# Autodesk Inventor assembly: YAxis
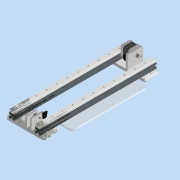
[picture p0: Inventor's stored thumbnail of the model, 180x180]
Saved by Autodesk Inventor 2022 (Build 260153000, 153)
## iProperties
Created: 2021-06-27
Part Number: YAxis
Document SubType Name: Assembly
Designer: domin
Author: domin
## Documents named in this file (19)
- D:\Sync\Hivemind\1-MCI-Unterlagen\Master\Semester 3\Projekt 2\011_Kartesischer_Roboter_Modul\07-CAD Files\02-Kartesischer Roboter\YAxis\YAxis.iam
- D:\Sync\Hivemind\1-MCI-Unterlagen\Master\Semester 3\Projekt 2\011_Kartesischer_Roboter_Modul\07-CAD Files\02-Kartesischer Roboter\Einzelteile\Fuehrungslager.ipt
- D:\Sync\Hivemind\1-MCI-Unterlagen\Master\Semester 3\Projekt 2\011_Kartesischer_Roboter_Modul\07-CAD Files\02-Kartesischer Roboter\Einzelteile\Y-Axis_back_plate_bottom.ipt
- D:\Sync\Hivemind\1-MCI-Unterlagen\Master\Semester 3\Projekt 2\011_Kartesischer_Roboter_Modul\07-CAD Files\02-Kartesischer Roboter\Einzelteile\Y-Axis_back_plate_top.ipt
- D:\Sync\Hivemind\1-MCI-Unterlagen\Master\Semester 3\Projekt 2\011_Kartesischer_Roboter_Modul\07-CAD Files\02-Kartesischer Roboter\Einzelteile\Y-Axis_front_plate_bottom.ipt
- D:\Sync\Hivemind\1-MCI-Unterlagen\Master\Semester 3\Projekt 2\011_Kartesischer_Roboter_Modul\07-CAD Files\02-Kartesischer Roboter\Einzelteile\Y-Axis_front_plate_top.ipt
- D:\Sync\Hivemind\1-MCI-Unterlagen\Master\Semester 3\Projekt 2\011_Kartesischer_Roboter_Modul\07-CAD Files\02-Kartesischer Roboter\Aluminum\X-Axis_motor_plate.ipt
- D:\Sync\Hivemind\1-MCI-Unterlagen\Master\Semester 3\Projekt 2\011_Kartesischer_Roboter_Modul\07-CAD Files\02-Kartesischer Roboter\Einzelteile\X-Kettenhalter2.ipt
- D:\Sync\Hivemind\1-MCI-Unterlagen\Master\Semester 3\Projekt 2\011_Kartesischer_Roboter_Modul\07-CAD Files\02-Kartesischer Roboter\Einzelteile\Y-Umlenkrollenhalter.ipt
- D:\Sync\Hivemind\1-MCI-Unterlagen\Master\Semester 3\Projekt 2\011_Kartesischer_Roboter_Modul\07-CAD Files\02-Kartesischer Roboter\Aluminum\X-Axis_beltplates.ipt
- D:\Sync\Hivemind\1-MCI-Unterlagen\Master\Semester 3\Projekt 2\011_Kartesischer_Roboter_Modul\07-CAD Files\02-Kartesischer Roboter\Einzelteile\Stift_5mm.ipt
- D:\Sync\Hivemind\1-MCI-Unterlagen\Master\Semester 3\Projekt 2\011_Kartesischer_Roboter_Modul\07-CAD Files\02-Kartesischer Roboter\Einzelteile\White_Cable_Tie_Mount_RS666-717.ipt
- D:\Sync\Hivemind\1-MCI-Unterlagen\Master\Semester 3\Projekt 2\011_Kartesischer_Roboter_Modul\07-CAD Files\02-Kartesischer Roboter\Einzelteile\Ender_Motor.ipt
- D:\Sync\Hivemind\1-MCI-Unterlagen\Master\Semester 3\Projekt 2\011_Kartesischer_Roboter_Modul\07-CAD Files\02-Kartesischer Roboter\Einzelteile\Endstop.ipt
- D:\Sync\Hivemind\1-MCI-Unterlagen\Master\Semester 3\Projekt 2\011_Kartesischer_Roboter_Modul\07-CAD Files\02-Kartesischer Roboter\Einzelteile\Umlenkrolle_5mm.ipt
- D:\Sync\Hivemind\1-MCI-Unterlagen\Master\Semester 3\Projekt 2\011_Kartesischer_Roboter_Modul\07-CAD Files\02-Kartesischer Roboter\Einzelteile\Zahnriemenscheibe_20teeth.ipt
- D:\Sync\Hivemind\1-MCI-Unterlagen\Master\Semester 3\Projekt 2\011_Kartesischer_Roboter_Modul\07-CAD Files\02-Kartesischer Roboter\ITEM_Profile\Schlitten_Profil.ipt
- D:\Sync\Hivemind\1-MCI-Unterlagen\Master\Semester 3\Projekt 2\011_Kartesischer_Roboter_Modul\07-CAD Files\02-Kartesischer Roboter\Einzelteile\Fuehrungsschiene440mm.ipt
- D:\Sync\Hivemind\1-MCI-Unterlagen\Master\Semester 3\Projekt 2\011_Kartesischer_Roboter_Modul\07-CAD Files\02-Kartesischer Roboter\Einzelteile\Y_Kettenhalter.ipt
## Components (25 placed, 18 different names)
1. Fuehrungslager:1 — Flush:2, Flush:3, Mate:1, Mate:2, Flush:4, Flush:5, Flush:6, Mate:3, Flush:7
2. Fuehrungslager:2 — Mate:2, Flush:4, Flush:5, Mate:5, Mate:6, Mate:7
3. Fuehrungslager:3 — Flush:6, Mate:3, Flush:7, Flush:8, Flush:9, Mate:4, Mate:9
4. Fuehrungslager:4 — Flush:8, Flush:9, Mate:4, Mate:10, Mate:11, Mate:47
5. Y-Axis_back_plate_bottom:1 — Mate:5, Mate:6, Mate:7, Mate:8, Flush:10, Flush:11
6. Y-Axis_back_plate_top:1 — Mate:8, Flush:10, Flush:11, Mate:13, Mate:14, Mate:15, Mate:16, Mate:17, Mate:18, Mate:40, Mate:42, Flush:17
7. Y-Axis_front_plate_bottom:1 — Mate:9, Mate:10, Mate:11, Mate:12, Flush:12, Flush:13
8. Y-Axis_front_plate_top:1 — Mate:12, Flush:12, Flush:13, Mate:19, Mate:20, Mate:21, Mate:22, Mate:23, Mate:24
9. X-Axis_motor_plate:1 — Mate:13, Mate:14, Mate:15, Mate:28, Mate:29, Mate:30, Mate:31, Mate:32, Mate:33, Flush:15
10. X-Kettenhalter2:1 — Mate:16, Mate:17, Mate:18, Mate:26, Mate:27, Angle:1, Mate:41
11. White_Cable_Tie_Mount_RS666-717:1 — Mate:26, Mate:27, Angle:1
12. Y-Umlenkrollenhalter:1 — Mate:19, Mate:20, Mate:21, Mate:25, Flush:14
13. X-Axis_beltplates:1 — Mate:22, Mate:23, Mate:24, Mate:34, Mate:36, Mate:37, Mate:38
14. Stift_5mm:1 — Mate:25, Flush:14, Mate:35
15. Ender_Motor:1 — Mate:28, Mate:29, Mate:30, Mate:39
16. Endstop:1 — Mate:31, Mate:32, Mate:33
17. Endstop:2 — Mate:36, Mate:37, Mate:38
18. Umlenkrolle_5mm:1 — Mate:34, Mate:35
19. Zahnriemenscheibe_20teeth:1 — Mate:39, Flush:15
20. Schlitten_Profil:1 — Mate:40, Mate:41, Mate:43, Flush:16, Flush:17, Mate:44, Flush:18, Flush:19, Mate:46, Flush:22, Mate:48, Mate:49
21. Schlitten_Profil:2 — Mate:42, Mate:43, Flush:16, Mate:45, Flush:20, Flush:21
22. Fuehrungsschiene440mm:1 — Mate:44, Flush:18, Flush:19
23. Fuehrungsschiene440mm:2 — Mate:45, Flush:20, Flush:21
24. Y_Kettenhalter:1 — Mate:46, Flush:22, Mate:47, Mate:50
25. White_Cable_Tie_Mount_RS666-717:2 — Mate:48, Mate:49, Mate:50
## Relationships (72: Mate 50, Flush 21, Angle 1)
- Flush:2: Fuehrungslager:1
- Flush:3: Fuehrungslager:1
- Mate:1: Fuehrungslager:1
- Mate:2 (36 mm): Fuehrungslager:1 ↔ Fuehrungslager:2
- Flush:4: Fuehrungslager:1 ↔ Fuehrungslager:2
- Flush:5: Fuehrungslager:1 ↔ Fuehrungslager:2
- Flush:6: Fuehrungslager:1 ↔ Fuehrungslager:3
- Mate:3 (358 mm): Fuehrungslager:1 ↔ Fuehrungslager:3
- Flush:7: Fuehrungslager:1 ↔ Fuehrungslager:3
- Flush:8: Fuehrungslager:3 ↔ Fuehrungslager:4
- Flush:9: Fuehrungslager:3 ↔ Fuehrungslager:4
- Mate:4 (36 mm): Fuehrungslager:3 ↔ Fuehrungslager:4
- Mate:5: Fuehrungslager:2 ↔ Y-Axis_back_plate_bottom:1
- Mate:6: Fuehrungslager:2 ↔ Y-Axis_back_plate_bottom:1
- Mate:7: Fuehrungslager:2 ↔ Y-Axis_back_plate_bottom:1
- Mate:8: Y-Axis_back_plate_bottom:1 ↔ Y-Axis_back_plate_top:1
- Flush:10: Y-Axis_back_plate_bottom:1 ↔ Y-Axis_back_plate_top:1
- Flush:11: Y-Axis_back_plate_bottom:1 ↔ Y-Axis_back_plate_top:1
- Mate:9: Fuehrungslager:3 ↔ Y-Axis_front_plate_bottom:1
- Mate:10: Fuehrungslager:4 ↔ Y-Axis_front_plate_bottom:1
- Mate:11: Fuehrungslager:4 ↔ Y-Axis_front_plate_bottom:1
- Mate:12: Y-Axis_front_plate_bottom:1 ↔ Y-Axis_front_plate_top:1
- Flush:12: Y-Axis_front_plate_bottom:1 ↔ Y-Axis_front_plate_top:1
- Flush:13: Y-Axis_front_plate_bottom:1 ↔ Y-Axis_front_plate_top:1
- Mate:13: Y-Axis_back_plate_top:1 ↔ X-Axis_motor_plate:1
- Mate:14: Y-Axis_back_plate_top:1 ↔ X-Axis_motor_plate:1
- Mate:15: Y-Axis_back_plate_top:1 ↔ X-Axis_motor_plate:1
- Mate:16: Y-Axis_back_plate_top:1 ↔ X-Kettenhalter2:1
- Mate:17: Y-Axis_back_plate_top:1 ↔ X-Kettenhalter2:1
- Mate:18: Y-Axis_back_plate_top:1 ↔ X-Kettenhalter2:1
- Mate:19: Y-Axis_front_plate_top:1 ↔ Y-Umlenkrollenhalter:1
- Mate:20: Y-Axis_front_plate_top:1 ↔ Y-Umlenkrollenhalter:1
- Mate:21: Y-Axis_front_plate_top:1 ↔ Y-Umlenkrollenhalter:1
- Mate:22: Y-Axis_front_plate_top:1 ↔ X-Axis_beltplates:1
- Mate:23: Y-Axis_front_plate_top:1 ↔ X-Axis_beltplates:1
- Mate:24: Y-Axis_front_plate_top:1 ↔ X-Axis_beltplates:1
- Mate:25: Y-Umlenkrollenhalter:1 ↔ Stift_5mm:1
- Flush:14 (-6 mm): Y-Umlenkrollenhalter:1 ↔ Stift_5mm:1
- Mate:26: X-Kettenhalter2:1 ↔ White_Cable_Tie_Mount_RS666-717:1
- Mate:27: X-Kettenhalter2:1 ↔ White_Cable_Tie_Mount_RS666-717:1
- Angle:1 (0 deg): X-Kettenhalter2:1 ↔ White_Cable_Tie_Mount_RS666-717:1
- Mate:28: X-Axis_motor_plate:1 ↔ Ender_Motor:1
- Mate:29: X-Axis_motor_plate:1 ↔ Ender_Motor:1
- Mate:30: X-Axis_motor_plate:1 ↔ Ender_Motor:1
- Mate:31: X-Axis_motor_plate:1 ↔ Endstop:1
- Mate:32: X-Axis_motor_plate:1 ↔ Endstop:1
- Mate:33: X-Axis_motor_plate:1 ↔ Endstop:1
- Mate:34 (1.5 mm): X-Axis_beltplates:1 ↔ Umlenkrolle_5mm:1
- Mate:35: Stift_5mm:1 ↔ Umlenkrolle_5mm:1
- Mate:36: X-Axis_beltplates:1 ↔ Endstop:2
- Mate:37: X-Axis_beltplates:1 ↔ Endstop:2
- Mate:38: X-Axis_beltplates:1 ↔ Endstop:2
- Mate:39: Ender_Motor:1 ↔ Zahnriemenscheibe_20teeth:1
- Flush:15 (-10 mm): X-Axis_motor_plate:1 ↔ Zahnriemenscheibe_20teeth:1
- Mate:40: Y-Axis_back_plate_top:1 ↔ Schlitten_Profil:1
- Mate:41 (1 mm): X-Kettenhalter2:1 ↔ Schlitten_Profil:1
- Mate:42: Y-Axis_back_plate_top:1 ↔ Schlitten_Profil:2
- Mate:43 (80 mm): Schlitten_Profil:1 ↔ Schlitten_Profil:2
- Flush:16: Schlitten_Profil:1 ↔ Schlitten_Profil:2
- Flush:17: Y-Axis_back_plate_top:1 ↔ Schlitten_Profil:1
- Mate:44: Schlitten_Profil:1 ↔ Fuehrungsschiene440mm:1
- Flush:18: Schlitten_Profil:1 ↔ Fuehrungsschiene440mm:1
- Flush:19: Schlitten_Profil:1 ↔ Fuehrungsschiene440mm:1
- Mate:45: Schlitten_Profil:2 ↔ Fuehrungsschiene440mm:2
- Flush:20: Schlitten_Profil:2 ↔ Fuehrungsschiene440mm:2
- Flush:21: Schlitten_Profil:2 ↔ Fuehrungsschiene440mm:2
- Mate:46: Schlitten_Profil:1 ↔ Y_Kettenhalter:1
- Flush:22: Schlitten_Profil:1 ↔ Y_Kettenhalter:1
- Mate:47 (34 mm): Fuehrungslager:4 ↔ Y_Kettenhalter:1
- Mate:48: Schlitten_Profil:1 ↔ White_Cable_Tie_Mount_RS666-717:2
- Mate:49: Schlitten_Profil:1 ↔ White_Cable_Tie_Mount_RS666-717:2
- Mate:50 (2.5 mm): Y_Kettenhalter:1 ↔ White_Cable_Tie_Mount_RS666-717:2
